# Autodesk Inventor assembly: BMS
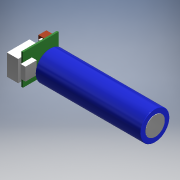
[picture p0: Inventor's stored thumbnail of the model, 180x180]
Saved by Autodesk Inventor 2019 (Build 230136000, 136)
## iProperties
Part Number: BMS
Document SubType Name: Assembly
Designer: usr
Author: usr
## Documents named in this file (3)
- C:\Users\usr\Documents\_Skola\Git-hub\Modular-Power-Bank\BMS.iam
- C:\Users\usr\Documents\_Skola\Git-hub\Modular-Power-Bank\Battery-Management.ipt
- C:\Users\usr\Documents\_Skola\Git-hub\Modular-Power-Bank\18650-battery.ipt
## Components (2 placed, 2 different names)
1. Battery-Management:1 — Rigid:1
2. 18650-battery:1 — Rigid:1
## Relationships (1: WeldJoint 1)
- Rigid:1 [WeldJoint] (5 mm): Battery-Management:1 ↔ 18650-battery:1
